# Autodesk Inventor assembly: motor
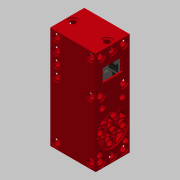
[picture p0: Inventor's stored thumbnail of the model, 180x180]
Saved by Autodesk Inventor 2019.3 (Build 233278000, 278)
## iProperties
Created: 2019-02-05
Part Number: motor
Document SubType Name: Assembly
Designer: Varga Daniel
Sending System: SolidWorks 2018
Last Author: david
Last Saved: 2019-02-15
Author: Varga Daniel
## Documents named in this file (7)
- C:\!_Dani\!_cloud\OneDrive\!_munka\Revolution\RevvyDemoKit\Structural parts\Demo parts\Motor\Inventor imported\motor.iam
- C:\!_Dani\!_cloud\OneDrive\!_munka\Revolution\RevvyDemoKit\Structural parts\Demo parts\Motor\Inventor imported\rj45_vert.ipt
- C:\!_Dani\!_cloud\OneDrive\!_munka\Revolution\RevvyDemoKit\Structural parts\Demo parts\Motor\Inventor imported\MOcA_1.ipt
- C:\!_Dani\!_cloud\OneDrive\!_munka\Revolution\RevvyDemoKit\Structural parts\Demo parts\Motor\Inventor imported\MOcA_2.ipt
- C:\!_Dani\!_cloud\OneDrive\!_munka\Revolution\RevvyDemoKit\Structural parts\Demo parts\Motor\Inventor imported\ff130-13200.ipt
- C:\!_Dani\!_cloud\OneDrive\!_munka\Revolution\RevvyDemoKit\Structural parts\Demo parts\Motor\Inventor imported\MOhA_2.ipt
- C:\!_Dani\!_cloud\OneDrive\!_munka\Revolution\RevvyDemoKit\Structural parts\Demo parts\Motor\Inventor imported\MOhA_1.ipt
## Components (6 placed, 6 different names)
1. rj45_vert:1 — Mate:2, Mate:4, Flush:5
2. MOhA_2:1 — Mate:5, Angle:1, Flush:4
3. MOhA_1:1 — Mate:1, Flush:1, Mate:5, Angle:1
4. MOcA_1:2 — Flush:2, Mate:6, Flush:3, Flush:4
5. MOcA_2:2 — Mate:1, Flush:1, Mate:2, Mate:4, Flush:2, Mate:6, Flush:3, Flush:5
6. ff130-13200:1
## Relationships (11: Mate 5, Flush 5, Angle 1)
- Mate:1: MOhA_1:1 ↔ MOcA_2:2
- Flush:1: MOhA_1:1 ↔ MOcA_2:2
- Mate:2: rj45_vert:1 ↔ MOcA_2:2
- Mate:4 (1.15 mm): rj45_vert:1 ↔ MOcA_2:2
- Mate:5: MOhA_2:1 ↔ MOhA_1:1
- Angle:1 (0 deg): MOhA_2:1 ↔ MOhA_1:1
- Flush:2: MOcA_1:2 ↔ MOcA_2:2
- Mate:6: MOcA_1:2 ↔ MOcA_2:2
- Flush:3: MOcA_1:2 ↔ MOcA_2:2
- Flush:4: MOhA_2:1 ↔ MOcA_1:2
- Flush:5: rj45_vert:1 ↔ MOcA_2:2
